# Autodesk Inventor assembly: Unit
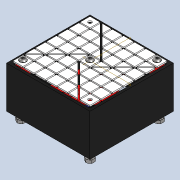
[picture p0: Inventor's stored thumbnail of the model, 180x180]
Saved by Autodesk Inventor 2022 (Build 260153000, 153)
## iProperties
Created: 2023-02-26
Part Number: Unit
Document SubType Name: Assembly
Designer: byrne
Author: byrne
## Documents named in this file (11)
- C:\Users\byrne\OneDrive\Documents\Inventor\RAI\Unit.iam
- C:\Users\byrne\OneDrive\Documents\Inventor\RAI\Frame.ipt
- C:\Users\byrne\OneDrive\Documents\Inventor\RAI\Pololu#1053 v4.ipt
- C:\Users\byrne\OneDrive\Documents\Inventor\RAI\Thingy.ipt
- C:\Users\byrne\OneDrive\Documents\Inventor\RAI\arm for thingy.ipt
- C:\Users\byrne\OneDrive\Documents\Inventor\RAI\Standoffs.ipt
- C:\Users\byrne\OneDrive\Documents\Inventor\RAI\93365A140_Tapered Heat-Set Inserts for Plastic.ipt
- C:\Users\byrne\OneDrive\Documents\Inventor\RAI\98164A134_316 Stainless Steel Button Head Hex Drive Screw.ipt
- C:\Users\byrne\OneDrive\Documents\Inventor\RAI\Flasher.ipt
- C:\Users\byrne\OneDrive\Documents\Inventor\RAI\98164A450_316 Stainless Steel Button Head Hex Drive Screw.ipt
- C:\Users\byrne\OneDrive\Documents\Inventor\RAI\90633A009_Low-Strength Steel Thin Nylon-Insert Locknut.ipt
## Components (30 placed, 10 different names)
1. Frame:1 — Mate:1, Mate:2, Mate:3, Angle:1, Tangent:1, Tangent:2, Tangent:3, Tangent:4, Mate:6, Mate:7, Insert:4, Mate:8, Mate:9, Insert:19, Insert:20, Insert:21, Insert:22, Insert:23, Insert:24, Insert:25, Insert:26
2. Pololu#1053 v4:1 — Mate:1, Mate:2, Mate:3, Angle:1, Insert:1
3. Thingy:1 — Insert:1, Insert:2, Insert:3, Insert:14, Insert:15
4. arm for thingy:1 — Insert:2, Tangent:1, Tangent:2, Mate:4, Insert:12, Insert:16
5. arm for thingy:2 — Insert:3, Tangent:3, Tangent:4, Mate:5, Insert:13, Insert:17
6. Standoffs:1 — Mate:5, Mate:7, Insert:6, Insert:7
7. Standoffs:2 — Mate:4, Mate:6, Insert:5, Insert:8
8. 93365A140_Tapered Heat-Set Inserts for Plastic:1 — Insert:6, Insert:11
9. 93365A140_Tapered Heat-Set Inserts for Plastic:2 — Insert:8
10. 93365A140_Tapered Heat-Set Inserts for Plastic:3 — Insert:4, Insert:10
11. 93365A140_Tapered Heat-Set Inserts for Plastic:4 — Insert:5, Insert:9
12. 93365A140_Tapered Heat-Set Inserts for Plastic:5 — Insert:7
13. 98164A134_316 Stainless Steel Button Head Hex Drive Screw:1 — Insert:9
14. 98164A134_316 Stainless Steel Button Head Hex Drive Screw:2 — Insert:10
15. 98164A134_316 Stainless Steel Button Head Hex Drive Screw:3 — Insert:12
16. 98164A134_316 Stainless Steel Button Head Hex Drive Screw:4 — Insert:13
17. 98164A134_316 Stainless Steel Button Head Hex Drive Screw:5 — Insert:11, Insert:18
18. 93365A140_Tapered Heat-Set Inserts for Plastic:6 — Insert:14
19. 93365A140_Tapered Heat-Set Inserts for Plastic:7 — Insert:15
20. 98164A134_316 Stainless Steel Button Head Hex Drive Screw:6 — Insert:16
21. 98164A134_316 Stainless Steel Button Head Hex Drive Screw:7 — Insert:17
22. Flasher:1 — Mate:8, Mate:9, Insert:18
23. 98164A450_316 Stainless Steel Button Head Hex Drive Screw:1 — Insert:22
24. 98164A450_316 Stainless Steel Button Head Hex Drive Screw:2 — Insert:21
25. 98164A450_316 Stainless Steel Button Head Hex Drive Screw:3 — Insert:20
26. 98164A450_316 Stainless Steel Button Head Hex Drive Screw:4 — Insert:19
27. 90633A009_Low-Strength Steel Thin Nylon-Insert Locknut:1 — Insert:25
28. 90633A009_Low-Strength Steel Thin Nylon-Insert Locknut:2 — Insert:23
29. 90633A009_Low-Strength Steel Thin Nylon-Insert Locknut:3 — Insert:24
30. 90633A009_Low-Strength Steel Thin Nylon-Insert Locknut:4 — Insert:26
## Relationships (40: Insert 26, Mate 9, Tangent 4, Angle 1)
- Mate:1 (47.625 mm): Frame:1 ↔ Pololu#1053 v4:1
- Mate:2 (47.625 mm): Frame:1 ↔ Pololu#1053 v4:1
- Mate:3: Frame:1 ↔ Pololu#1053 v4:1
- Angle:1 (0 deg): Frame:1 ↔ Pololu#1053 v4:1
- Insert:1: Pololu#1053 v4:1 ↔ Thingy:1
- Insert:2: Thingy:1 ↔ arm for thingy:1
- Insert:3: Thingy:1 ↔ arm for thingy:2
- Tangent:1 (0.254 mm): Frame:1 ↔ arm for thingy:1
- Tangent:2 (0.254 mm): Frame:1 ↔ arm for thingy:1
- Tangent:3 (0.254 mm): Frame:1 ↔ arm for thingy:2
- Tangent:4 (0.254 mm): Frame:1 ↔ arm for thingy:2
- Mate:4: arm for thingy:1 ↔ Standoffs:2
- Mate:5: arm for thingy:2 ↔ Standoffs:1
- Mate:6: Frame:1 ↔ Standoffs:2
- Mate:7: Frame:1 ↔ Standoffs:1
- Insert:4: Frame:1 ↔ 93365A140_Tapered Heat-Set Inserts for Plastic:3
- Insert:5: Standoffs:2 ↔ 93365A140_Tapered Heat-Set Inserts for Plastic:4
- Insert:6: Standoffs:1 ↔ 93365A140_Tapered Heat-Set Inserts for Plastic:1
- Insert:7: Standoffs:1 ↔ 93365A140_Tapered Heat-Set Inserts for Plastic:5
- Insert:8: Standoffs:2 ↔ 93365A140_Tapered Heat-Set Inserts for Plastic:2
- Insert:9 (3.175 mm): 93365A140_Tapered Heat-Set Inserts for Plastic:4 ↔ 98164A134_316 Stainless Steel Button Head Hex Drive Screw:1
- Insert:10 (3.175 mm): 93365A140_Tapered Heat-Set Inserts for Plastic:3 ↔ 98164A134_316 Stainless Steel Button Head Hex Drive Screw:2
- Insert:11 (3.175 mm): 93365A140_Tapered Heat-Set Inserts for Plastic:1 ↔ 98164A134_316 Stainless Steel Button Head Hex Drive Screw:5
- Insert:12: arm for thingy:1 ↔ 98164A134_316 Stainless Steel Button Head Hex Drive Screw:3
- Insert:13: arm for thingy:2 ↔ 98164A134_316 Stainless Steel Button Head Hex Drive Screw:4
- Insert:14: Thingy:1 ↔ 93365A140_Tapered Heat-Set Inserts for Plastic:6
- Insert:15: Thingy:1 ↔ 93365A140_Tapered Heat-Set Inserts for Plastic:7
- Insert:16: arm for thingy:1 ↔ 98164A134_316 Stainless Steel Button Head Hex Drive Screw:6
- Insert:17: arm for thingy:2 ↔ 98164A134_316 Stainless Steel Button Head Hex Drive Screw:7
- Mate:8: Frame:1 ↔ Flasher:1
- Mate:9 (0.7937 mm): Frame:1 ↔ Flasher:1
- Insert:18 (0.7937 mm): 98164A134_316 Stainless Steel Button Head Hex Drive Screw:5 ↔ Flasher:1
- Insert:19: Frame:1 ↔ 98164A450_316 Stainless Steel Button Head Hex Drive Screw:4
- Insert:20: Frame:1 ↔ 98164A450_316 Stainless Steel Button Head Hex Drive Screw:3
- Insert:21: Frame:1 ↔ 98164A450_316 Stainless Steel Button Head Hex Drive Screw:2
- Insert:22: Frame:1 ↔ 98164A450_316 Stainless Steel Button Head Hex Drive Screw:1
- Insert:23 (6.35 mm): Frame:1 ↔ 90633A009_Low-Strength Steel Thin Nylon-Insert Locknut:2
- Insert:24 (6.35 mm): Frame:1 ↔ 90633A009_Low-Strength Steel Thin Nylon-Insert Locknut:3
- Insert:25 (6.35 mm): Frame:1 ↔ 90633A009_Low-Strength Steel Thin Nylon-Insert Locknut:1
- Insert:26 (6.35 mm): Frame:1 ↔ 90633A009_Low-Strength Steel Thin Nylon-Insert Locknut:4
